# Autodesk Inventor assembly: Motor Stand Assembly
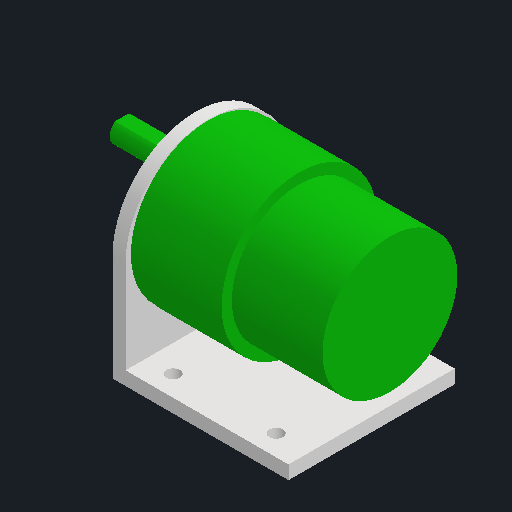
[picture p0: Inventor's stored thumbnail of the model, 512x512]
Saved by Autodesk Inventor 2026.2 (Build 302298010, 298A)
## iProperties
Created: 2026-06-06
Part Number: Motor Stand Assembly
Document SubType Name: Assembly
Designer: Inigo Greenall
Author: Inigo Greenall
## Documents named in this file (3)
- C:\Users\Inigo Greenall\OneDrive\Excavator Project\Motor\Motor Stand Assembly.iam
- C:\Users\Inigo Greenall\OneDrive\Excavator Project\Motor\Drive Motor Stand.ipt
- C:\Users\Inigo Greenall\OneDrive\Excavator Project\Motor\Drive Motor approximate.ipt
## Components (2 placed, 2 different names)
1. Drive Motor Stand:1 — Mate:1, Mate:2
2. Drive Motor approximate:1 — Mate:1, Mate:2
## Relationships (2: Mate 2)
- Mate:1: Drive Motor Stand:1 ↔ Drive Motor approximate:1
- Mate:2: Drive Motor Stand:1 ↔ Drive Motor approximate:1
